# Autodesk Inventor assembly: C-SV2R24-160
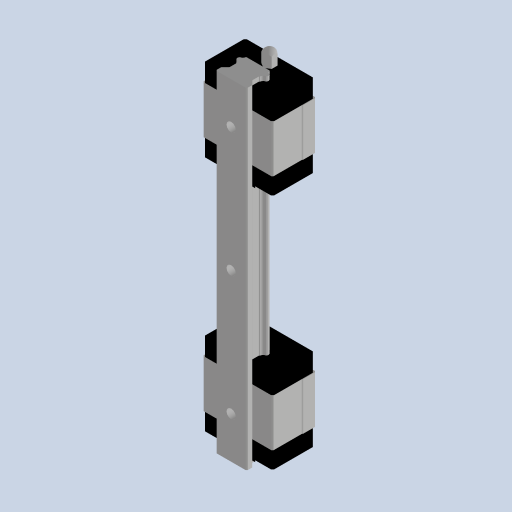
[picture p0: Inventor's stored thumbnail of the model, 512x512]
Saved by Autodesk Inventor 2023 (Build 270158000, 158)
## iProperties
Category: PARTsolutions
Company: MISUMI
Created: 2024-12-12
Part Number: C-SV2R24-160
Catalog Web Link: www.cadenas.de
Description: C-SVR, C-SV2R, C-SVRL, C-SV2RL-C-VALUE Linear Guides for Medium Load
Vendor: MISUMI
Document SubType Name: Assembly
Designer: psAdmin
Manufacturer: MISUMI
Mass: 70.6246 g
Surface Area: 232.458 cm^2
Volume: 70.6246 cm^3
Density: 1 g/cm^3
PSOL_IDENT_0: {$CADENAS_DATA/23d-libs/misumi/metric/06_linear_guides/06_cn/c_svr_asmtab.prj},217 {VTYP=3D},{STYP=A
PSOL_IDENT_1: SSTAB},{NB=C-SV2R24-160},{LINA=C-SV2R24-160},{NN=C-SVR, C-SV2R, C-SVRL, C-SV2RL},{DATE=21.04.2022 05
PSOL_IDENT_2: :41:22},{GEOMDATE=11.06.2020 07:59:43},{VERSION=},{LINEID=10},{WBVAR=NOB,LT,LS,ALT},{WBNUMERIC=LS}
PSOL_IDENT_3: {NB=C-SV2R24-160},{LINA=C-SV2R24-160},{KT=DUMMY},{PN=C-SV2R24-160},{TYPE=C-SV},{H=24},{NOB=2},{LT=},
PSOL_IDENT_4: {LS=160},{LALG=[160,220,280,340,400,460,520,580,640,700,760,820,880,940,1000,1060,1120,1180,1240,130
PSOL_IDENT_5: 0,1360,1420,1480]},{LSALG=[160,220,280,340,400,460,520,580,640,700,760,820,880,940,1000,1060,1120,11
PSOL_IDENT_6: 80,1240,1300,1360,1420,1480]},{LALG0=[170:210/10],[230:270/10],[290:330/10],[350:390/10],[410:450/10
PSOL_IDENT_7: ],[470:510/10],[530:570/10],[590:630/10],[650:690/10],[710:750/10],[770:810/10],[830:870/10],[890:93
PSOL_IDENT_8: 0/10],[950:990/10],[1010:1050/10],[1070:1110/10],[1130:1170/10],[1190:1230/10],[1250:1290/10],[1310:
PSOL_IDENT_9: 1350/10],[1370:1410/10],[1430:1470/10]},{LMIN=170},{LMAX=1470},{W=34},{L1=39.3},{B=26},{S=4.000},{LL=
PSOL_IDENT_10: 5.000},{SLL=M4x5},{L2=22.9},{K=20.8},{T=6.20},{CBB=0.5},{E=7},{T1=5.5},{H1=13.0},{W1=15},{W2=9.5},{C
PSOL_IDENT_11: AA=0.5},{DD1=4.5},{DD2=7.5},{HH=6.0},{DDH=4.5x7.5x6},{F=60},{G=20},{LW1=7.217},{LW2=11.000},{LH1=8.2
PSOL_IDENT_12: 21},{LH2=4.659},{LH3=3.221},{LH4=4.700},{LR1=1.431},{LR2=0.300},{LR3=0.300},{LR4=0.300},{M=3},{ALT=}
PSOL_IDENT_13: ,{ALTALG= '','N/A' },{NL=40},{PPATH=c_svr/c_svr_asmtpl.prj}
NB: C-SV2R24-160
NN: C-SVR, C-SV2R, C-SVRL, C-SV2RL
NT: C-VALUE Linear Guides for Medium Load
NBSYN: $PN.
LINA: C-SV2R24-160
CATALOG: Misumi
PN: C-SV2R24-160
H: 24
NOB: 2
LT: Selectable
LS: 160
W: 34
L1: 39.3
B: 26
SLL: M4x5
L2: 22.9
K: 20.8
T: 6.2
CBB: 0.5
E: 7
T1: 5.5
H1: 13
W1: 15
W2: 9.5
CAA: 0.5
DDH: 4.5x7.5x6
F: 60
G: 20
ALT: N/A
SUPPLIER: MISUMI
ARTICLENO: C-SV2R24-160
BOMINFO: C-SV2R24-160
CREATOR: CADENAS GmbH
Title: C-SV2R24-160
Author: Cadenas PARTsolutions
Comments: C-VALUE Linear Guides for Medium Load
## Documents named in this file (4)
- D:\GitHub\inventor\syu-si\OfficeRobot\ReadyMade\linear_guide\C-SV2R24-160.iam
- D:\GitHub\inventor\syu-si\OfficeRobot\ReadyMade\linear_guide\C-SV2R24-160_r.ipt
- D:\GitHub\inventor\syu-si\OfficeRobot\ReadyMade\linear_guide\C-SV2R24-L_b.ipt
- D:\GitHub\inventor\syu-si\OfficeRobot\ReadyMade\linear_guide\C-SV2R24-R_b.ipt
## Components (3 placed, 3 different names)
1. C-SV2R24-160_r:1 — to_block_1_Z@1 <-> to_rail_Z@2, to_block_1_YZ@1 <-> to_rail_YZ@2, to_block_2_Z@1 <-> to_rail_Z@3, to_block_2_YZ@1 <-> to_rail_YZ@3
2. C-SV2R24-L_b:1 — to_block_1_Z@1 <-> to_rail_Z@2, to_block_1_YZ@1 <-> to_rail_YZ@2
3. C-SV2R24-R_b:1 — to_block_2_Z@1 <-> to_rail_Z@3, to_block_2_YZ@1 <-> to_rail_YZ@3
## Relationships (4: Mate 2, Angle 2)
- to_block_1_Z@1 <-> to_rail_Z@2 [Mate]: C-SV2R24-160_r:1 ↔ C-SV2R24-L_b:1
- to_block_1_YZ@1 <-> to_rail_YZ@2 [Angle] (180 deg): C-SV2R24-160_r:1 ↔ C-SV2R24-L_b:1
- to_block_2_Z@1 <-> to_rail_Z@3 [Mate]: C-SV2R24-160_r:1 ↔ C-SV2R24-R_b:1
- to_block_2_YZ@1 <-> to_rail_YZ@3 [Angle] (180 deg): C-SV2R24-160_r:1 ↔ C-SV2R24-R_b:1
